# Autodesk Inventor assembly: 8 inch mecanum with toughbox (Right)
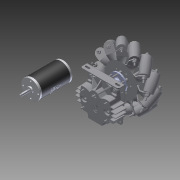
[picture p0: Inventor's stored thumbnail of the model, 180x180]
Saved by Autodesk Inventor 2014 (Build 180170000, 170)
## iProperties
Created: 2015-01-10
Part Number: 8 inch mecanum with toughbox (Right)
Document SubType Name: Assembly
Designer: student
Author: student
## Documents named in this file (6)
- C:\Users\student\Documents\Inventor\2015 Recycle Rush\8 inch mecanum with toughbox (Right).iam
- C:\Users\student\Documents\Inventor\2015 Recycle Rush\8 inch mecanum left wheel_MIR.iam
- C:\Users\student\Documents\Inventor\2015 Recycle Rush\am-0077a-500 Key Hub r2_MIR.ipt
- C:\Users\student\Documents\Inventor\2015 Recycle Rush\Derived Toughbox mini_MIR.ipt
- C:\Users\student\Documents\Inventor\Dillon And Justin\Imported Components\MOT_CIM-Motor_217-2000.iam\MOT_CIM-Motor_217-2000.iam.iam
- MOT_CIM-Motor_217-2000.iam
## Components (4 placed, 4 different names)
1. 8 inch mecanum left wheel_MIR:1 [sub-assembly] — Mate:1, Mate:2, Mate:3, Mate:5
2. am-0077a-500 Key Hub r2_MIR:1 — Mate:1, Mate:2, Mate:3, Mate:4, Mate:6
3. Derived Toughbox mini_MIR:1 — Mate:4, Angle:1, Mate:6
4. MOT_CIM-Motor_217-2000.iam:1 [sub-assembly]
## Relationships (7: Mate 6, Angle 1)
- Mate:1: 8 inch mecanum left wheel_MIR:1 ↔ am-0077a-500 Key Hub r2_MIR:1
- Mate:2: 8 inch mecanum left wheel_MIR:1 ↔ am-0077a-500 Key Hub r2_MIR:1
- Mate:3: 8 inch mecanum left wheel_MIR:1 ↔ am-0077a-500 Key Hub r2_MIR:1
- Mate:4: am-0077a-500 Key Hub r2_MIR:1 ↔ Derived Toughbox mini_MIR:1
- Angle:1 (0 deg): Derived Toughbox mini_MIR:1
- Mate:5: 8 inch mecanum left wheel_MIR:1
- Mate:6: am-0077a-500 Key Hub r2_MIR:1 ↔ Derived Toughbox mini_MIR:1
